# Autodesk Inventor assembly: アーム用3段
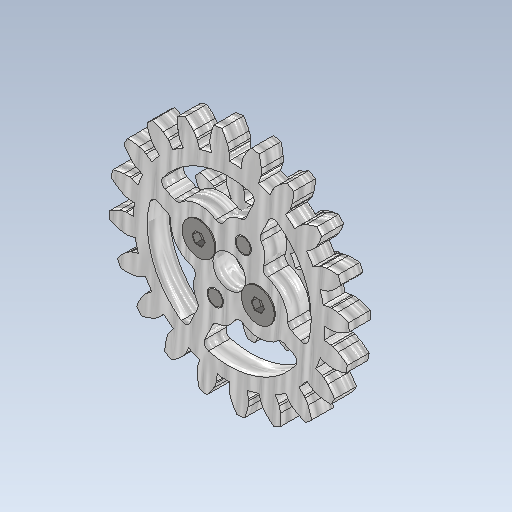
[picture p0: Inventor's stored thumbnail of the model, 512x512]
Saved by Autodesk Inventor 2020.2 (Build 242310000, 310)
## iProperties
Created: 2020-03-16
Part Number: アーム用3段
Document SubType Name: Assembly
Designer: aoyam
Mass: 16.5223 g
Surface Area: 58.5021 cm^2
Volume: 5.32439 cm^3
Density: 3.10313 g/cm^3
Author: aoyam
## Documents named in this file (5)
- C:\Users\aoyam\Desktop\SRDC_local\Inventor\二年機\Geminiβ\腕\アーム用3段.iam
- C:\Users\aoyam\Desktop\SRDC_local\Inventor\二年機\Geminiβ\汎用部品\ｍ2歯数11ギア6td5.98.ipt
- C:\Users\aoyam\Desktop\SRDC_local\Inventor\二年機\Geminiβ\汎用部品\ｍ2歯数20ギアd5.98.ipt
- C:\Users\aoyam\Desktop\SRDC_local\Inventor\二年機\Geminiβ\汎用部品\平行ピンD3L10.ipt
- C:\Users\aoyam\Desktop\SRDC_local\Inventor\二年機\Geminiβ\汎用部品\ネジ皿M3L8.ipt
## Components (6 placed, 4 different names)
1. ｍ2歯数11ギア6td5.98:1 — 挿入:1, メイト:1
2. ｍ2歯数20ギアd5.98:1 — 挿入:1, メイト:1, 挿入:2, 挿入:3, 挿入:4, 挿入:5
3. 平行ピンD3L10:1 — 挿入:2
4. 平行ピンD3L10:2 — 挿入:3
5. ネジ皿M3L8:1 — 挿入:5
6. ネジ皿M3L8:2 — 挿入:4
## Relationships (6: Insert 5, Mate 1)
- 挿入:1 [Insert]: ｍ2歯数11ギア6td5.98:1 ↔ ｍ2歯数20ギアd5.98:1
- メイト:1 [Mate]: ｍ2歯数11ギア6td5.98:1 ↔ ｍ2歯数20ギアd5.98:1
- 挿入:2 [Insert]: ｍ2歯数20ギアd5.98:1 ↔ 平行ピンD3L10:1
- 挿入:3 [Insert]: ｍ2歯数20ギアd5.98:1 ↔ 平行ピンD3L10:2
- 挿入:4 [Insert]: ｍ2歯数20ギアd5.98:1 ↔ ネジ皿M3L8:2
- 挿入:5 [Insert]: ｍ2歯数20ギアd5.98:1 ↔ ネジ皿M3L8:1
